# Autodesk Inventor assembly: CatapultAssembly
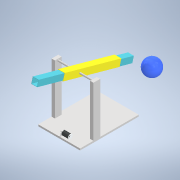
[picture p0: Inventor's stored thumbnail of the model, 180x180]
Saved by Autodesk Inventor 2022.2 (Build 262287000, 287)
## iProperties
Created: 2022-01-16
Part Number: CatapultAssembly
Document SubType Name: Assembly
Designer: robst
Author: robst
## Documents named in this file (8)
- C:\git\CAD-Development\robSteele\2022 Robot\CatapultAssembly.iam
- C:\git\CAD-Development\robSteele\2022 Robot\Catapult.ipt
- C:\git\CAD-Development\robSteele\2022 Robot\CatapultArm.ipt
- C:\git\CAD-MfgResources\Andy-Mark\Motors\am-0255 2.5inch CIM Motor.ipt
- C:\git\CAD-Development\robSteele\2022 Robot\CatapultArmExtensionForRear.ipt
- C:\git\CAD-Development\robSteele\2022 Robot\CatapultArmExtensionForFront.ipt
- C:\git\CAD-Development\robSteele\2022 Robot\BlueCargo.ipt
- C:\git\CAD-Development\robSteele\2022 Robot\am-4244 1IN Bent Bearing Side Mount Gusset.ipt
## Components (7 placed, 7 different names)
1. Catapult:1 — Mate:1, Mate:9, Flush:2
2. CatapultArm:1 — Mate:1, Mate:2, Mate:3, Mate:4, Mate:5, Flush:1, Mate:6, Mate:7
3. am-0255 2.5inch CIM Motor:1 — Insert:1
4. CatapultArmExtensionForRear:1 — Mate:3, Mate:4, Mate:5
5. CatapultArmExtensionForFront:1 — Flush:1, Mate:6, Mate:7
6. BlueCargo:1
7. am-4244 1IN Bent Bearing Side Mount Gusset:1 — Mate:8, Mate:9, Flush:2, Insert:1
## Relationships (12: Mate 9, Flush 2, Insert 1)
- Mate:1: Catapult:1 ↔ CatapultArm:1
- Mate:2: CatapultArm:1
- Mate:3 (-406.4 mm): CatapultArm:1 ↔ CatapultArmExtensionForRear:1
- Mate:4: CatapultArm:1 ↔ CatapultArmExtensionForRear:1
- Mate:5: CatapultArm:1 ↔ CatapultArmExtensionForRear:1
- Flush:1 (203.2 mm): CatapultArm:1 ↔ CatapultArmExtensionForFront:1
- Mate:6: CatapultArm:1 ↔ CatapultArmExtensionForFront:1
- Mate:7: CatapultArm:1 ↔ CatapultArmExtensionForFront:1
- Mate:8: am-4244 1IN Bent Bearing Side Mount Gusset:1
- Mate:9: Catapult:1 ↔ am-4244 1IN Bent Bearing Side Mount Gusset:1
- Flush:2: Catapult:1 ↔ am-4244 1IN Bent Bearing Side Mount Gusset:1
- Insert:1: am-0255 2.5inch CIM Motor:1 ↔ am-4244 1IN Bent Bearing Side Mount Gusset:1
